# Autodesk Inventor assembly: roller cage
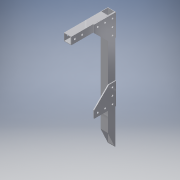
[picture p0: Inventor's stored thumbnail of the model, 180x180]
Saved by Autodesk Inventor 2016 (Build 200138000, 138)
## iProperties
Created: 2016-02-02
Part Number: roller cage
Document SubType Name: Assembly
Designer: gus
Mass: 119.442 g
Surface Area: 1363.6 cm^2
Volume: 119.442 cm^3
Density: 1 g/cm^3
Author: gus
## Documents named in this file (4)
- C:\Users\zachary\Downloads\robotfeb03\1510-stronghold-CAD-master\roller cage\roller cage.iam
- C:\Users\zachary\Downloads\robotfeb03\1510-stronghold-CAD-master\roller cage\top.ipt
- C:\Users\zachary\Downloads\robotfeb03\1510-stronghold-CAD-master\roller cage\vertical support.ipt
- C:\Users\zachary\Downloads\robotfeb03\1510-stronghold-CAD-master\roller cage\gusset plate.ipt
## Components (4 placed, 3 different names)
1. top:1 — Flush:1, Flush:2, Mate:1, Mate:2, Flush:4, Flush:5, Mate:3
2. vertical support:1 — Flush:1, Flush:2, Mate:1, Flush:3
3. gusset plate:1 — Mate:2, Flush:3, Flush:4
4. gusset plate:2 — Flush:5, Mate:3
## Relationships (8: Flush 5, Mate 3)
- Flush:1: top:1 ↔ vertical support:1
- Flush:2: top:1 ↔ vertical support:1
- Mate:1: top:1 ↔ vertical support:1
- Mate:2: top:1 ↔ gusset plate:1
- Flush:3: vertical support:1 ↔ gusset plate:1
- Flush:4: top:1 ↔ gusset plate:1
- Flush:5: top:1 ↔ gusset plate:2
- Mate:3: top:1 ↔ gusset plate:2
